# Autodesk Inventor assembly: table
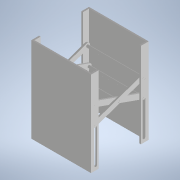
[picture p0: Inventor's stored thumbnail of the model, 180x180]
Saved by Autodesk Inventor 2020 (Build 240168000, 168)
## iProperties
Created: 2019-12-21
Part Number: table
Document SubType Name: Assembly
Designer: damien
Author: damien
## Documents named in this file (6)
- D:\fablab\save\Scisor\table.iam
- D:\fablab\save\Scisor\Plate.ipt
- D:\fablab\save\Scisor\rail.ipt
- D:\fablab\save\Scisor\rod.ipt
- D:\fablab\save\Scisor\foot.ipt
- D:\fablab\save\Scisor\center_rod.ipt
## Components (15 placed, 5 different names)
1. Plate:1 — Affleurement:1, Affleurement:2, Affleurement:3, Affleurement:4, Affleurement:5, Affleurement:6, Affleurement:7, Placage:29, Placage:30
2. rail:1 — Affleurement:4, Affleurement:5, Placage:3, Placage:4, Placage:30, Tangente:3
3. rail:2 — Affleurement:6, Affleurement:7, Affleurement:8, Affleurement:9, Placage:14, Placage:29, Tangente:4
4. rod:1 — Affleurement:8, Placage:3, Placage:5, Placage:12
5. rod:2 — Affleurement:9, Placage:4, Placage:7, Placage:13, Tangente:3, Tangente:4
6. foot:1 — Placage:7, Placage:9, Placage:33, Placage:34
7. foot:2 — Placage:5, Placage:9, Placage:33
8. foot:3 — Placage:10, Placage:11, Placage:12, Placage:26
9. foot:4 — Placage:10, Placage:11, Placage:13, Placage:14, Placage:24, Placage:25, Placage:32, Affleurement:21
10. rod:4 — Affleurement:16, Placage:17, Placage:25
11. rod:5 — Affleurement:18, Placage:23, Placage:26, Tangente:1, Tangente:2
12. Plate:2 — Affleurement:12, Affleurement:19, Affleurement:20, Placage:31, Placage:35
13. rail:3 — Affleurement:12, Affleurement:16, Placage:17, Affleurement:18, Placage:24, Placage:31, Tangente:2
14. rail:4 — Affleurement:19, Affleurement:20, Placage:23, Tangente:1, Placage:34, Placage:35
15. center_rod:1 — Placage:32, Affleurement:21
## Relationships (41: Mate 22, Flush 15, Tangent 4)
- Affleurement:1 [Flush]: Plate:1
- Affleurement:2 [Flush]: Plate:1
- Affleurement:3 [Flush]: Plate:1
- Affleurement:4 [Flush]: Plate:1 ↔ rail:1
- Affleurement:5 [Flush]: Plate:1 ↔ rail:1
- Affleurement:6 [Flush]: Plate:1 ↔ rail:2
- Affleurement:7 [Flush]: Plate:1 ↔ rail:2
- Affleurement:8 [Flush]: rail:2 ↔ rod:1
- Placage:3 [Mate]: rail:1 ↔ rod:1
- Affleurement:9 [Flush]: rail:2 ↔ rod:2
- Placage:4 [Mate]: rail:1 ↔ rod:2
- Placage:5 [Mate]: rod:1 ↔ foot:2
- Placage:7 [Mate]: rod:2 ↔ foot:1
- Placage:9 [Mate]: foot:1 ↔ foot:2
- Placage:10 [Mate]: foot:3 ↔ foot:4
- Placage:11 [Mate]: foot:3 ↔ foot:4
- Placage:12 [Mate]: rod:1 ↔ foot:3
- Placage:13 [Mate]: rod:2 ↔ foot:4
- Placage:14 [Mate]: rail:2 ↔ foot:4
- Affleurement:12 [Flush]: Plate:2 ↔ rail:3
- Affleurement:16 [Flush]: rod:4 ↔ rail:3
- Placage:17 [Mate]: rod:4 ↔ rail:3
- Affleurement:18 [Flush]: rod:5 ↔ rail:3
- Affleurement:19 [Flush]: Plate:2 ↔ rail:4
- Affleurement:20 [Flush]: Plate:2 ↔ rail:4
- Placage:23 [Mate]: rod:5 ↔ rail:4
- Placage:24 [Mate]: foot:4 ↔ rail:3
- Placage:25 [Mate]: foot:4 ↔ rod:4
- Placage:26 [Mate]: foot:3 ↔ rod:5
- Placage:29 [Mate]: Plate:1 ↔ rail:2
- Placage:30 [Mate]: Plate:1 ↔ rail:1
- Placage:31 [Mate]: Plate:2 ↔ rail:3
- Tangente:1: rod:5 ↔ rail:4
- Tangente:2: rod:5 ↔ rail:3
- Tangente:3: rail:1 ↔ rod:2
- Tangente:4: rail:2 ↔ rod:2
- Placage:32 [Mate]: foot:4 ↔ center_rod:1
- Affleurement:21 [Flush]: foot:4 ↔ center_rod:1
- Placage:33 [Mate]: foot:1 ↔ foot:2
- Placage:34 [Mate]: foot:1 ↔ rail:4
- Placage:35 [Mate]: Plate:2 ↔ rail:4
